# Autodesk Inventor assembly: mascon-new
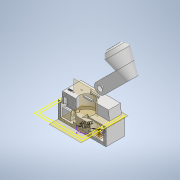
[picture p0: Inventor's stored thumbnail of the model, 180x180]
Saved by Autodesk Inventor 2021 (Build 250183000, 183)
## iProperties
Created: 2021-04-28
Part Number: mascon-new
Document SubType Name: Assembly
Designer: ben
Author: ben
## Documents named in this file (11)
- C:\Users\teh18\OneDrive\BVE Controller\r68-bve-mascon\mascon-new.iam
- C:\Users\teh18\OneDrive\BVE Controller\r68-bve-mascon\mascon.ipt
- C:\Users\teh18\OneDrive\BVE Controller\r68-bve-mascon\handle_base2.ipt
- C:\Users\teh18\OneDrive\BVE Controller\r68-bve-mascon\stl2\NotchPiston1.ipt
- C:\Users\teh18\OneDrive\BVE Controller\r68-bve-mascon\stl2\HandleBaseFiller.ipt
- C:\Users\teh18\OneDrive\BVE Controller\r68-bve-mascon\handle-stick.ipt
- C:\Users\teh18\OneDrive\BVE Controller\r68-bve-mascon\handle-sheath.ipt
- C:\Users\teh18\OneDrive\BVE Controller\r68-bve-mascon\stl2\Handle.iam
- C:\Users\teh18\OneDrive\BVE Controller\potentiometer-b10k-1.snapshot.2\PotentiometerB10K.ipt
- C:\Users\teh18\OneDrive\BVE Controller\r68-bve-mascon\PotHolder.ipt
- C:\Users\teh18\OneDrive\BVE Controller\r68-bve-mascon\stl2\HandleBaseFiller_MIR.ipt
## Components (10 placed, 10 different names)
1. mascon:1 — Flush:3, Mate:3, Mate:4, Tangent:1
2. handle_base2:1
3. NotchPiston1:1 — Flush:3
4. handle-sheath:1 — Mate:1, Mate:6
5. handle-stick:1 — Mate:1, Mate:6
6. HandleBaseFiller:1
7. Handle:1 [sub-assembly]
8. PotentiometerB10K:1 — Mate:4, Tangent:1
9. PotHolder:1 — Mate:3
10. HandleBaseFiller_MIR:1
## Relationships (6: Mate 4, Flush 1, Tangent 1)
- Flush:3: mascon:1 ↔ NotchPiston1:1
- Mate:1: handle-sheath:1 ↔ handle-stick:1
- Mate:3: mascon:1 ↔ PotHolder:1
- Mate:4: mascon:1 ↔ PotentiometerB10K:1
- Tangent:1: mascon:1 ↔ PotentiometerB10K:1
- Mate:6: handle-sheath:1 ↔ handle-stick:1
